# Autodesk Inventor assembly: Weldment
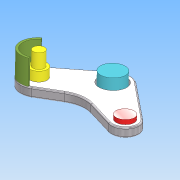
[picture p0: Inventor's stored thumbnail of the model, 180x180]
Saved by Autodesk Inventor 2020.1 (Build 241239000, 239)
## iProperties
Created: 2019-09-05
Part Number: Weldment
Document SubType Name: Assembly
Designer: thom_tremblay
Author: thom_tremblay
## Documents named in this file (6)
- C:\Users\thom_tremblay\Desktop\Inventor ACP Data\Weldment.iam
- C:\Users\thom_tremblay\Desktop\Inventor ACP Data\Parts\WeldExer_base.ipt
- C:\Users\thom_tremblay\Desktop\Inventor ACP Data\Parts\WeldExer_sleeve.ipt
- C:\Users\thom_tremblay\Desktop\Inventor ACP Data\Parts\WeldExer_upper_sleeve.ipt
- C:\Users\thom_tremblay\Desktop\Inventor ACP Data\Parts\WeldExer_lower_sleeve.ipt
- C:\Users\thom_tremblay\Desktop\Inventor ACP Data\Parts\WeldExer_Guard_Plate.ipt
## Components (5 placed, 5 different names)
1. WeldExer_base:1 — Insert:1, Insert:2, Insert:3, Insert:4, Angle:1
2. WeldExer_sleeve:1 — Insert:1
3. WeldExer_upper_sleeve:1 — Insert:2
4. WeldExer_lower_sleeve:1 — Insert:3
5. WeldExer_Guard_Plate:1 — Insert:4, Angle:1
## Relationships (5: Insert 4, Angle 1)
- Insert:1 (4.5 mm): WeldExer_base:1 ↔ WeldExer_sleeve:1
- Insert:2: WeldExer_base:1 ↔ WeldExer_upper_sleeve:1
- Insert:3: WeldExer_base:1 ↔ WeldExer_lower_sleeve:1
- Insert:4: WeldExer_base:1 ↔ WeldExer_Guard_Plate:1
- Angle:1 (0 deg): WeldExer_base:1 ↔ WeldExer_Guard_Plate:1
